# Autodesk Inventor assembly: LongAxisCradle
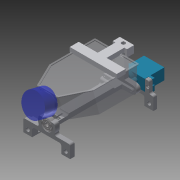
[picture p0: Inventor's stored thumbnail of the model, 180x180]
Saved by Autodesk Inventor 2014 SP1 (Build 180222100, 222)
## iProperties
Created: 2017-05-20
Part Number: LongAxisCradle
Document SubType Name: Assembly
Designer: danielsikar
Author: danielsikar
## Documents named in this file (9)
- C:\Users\danielsikar\Documents\Inventor\FlaskCradle\assemblies\LongAxisCradle.iam
- C:\Users\danielsikar\Documents\Inventor\FlaskCradle\parts\Flask.ipt
- C:\Users\danielsikar\Documents\Inventor\FlaskCradle\assemblies\ServoAndHorn.iam
- C:\Users\danielsikar\Documents\Inventor\FlaskCradle\parts\Bearing-605zz.ipt
- C:\Users\danielsikar\Documents\Inventor\FlaskCradle\parts\LongAxisShaft.ipt
- C:\Users\danielsikar\Documents\Inventor\FlaskCradle\parts\LongAxisTopClamp.ipt
- C:\Users\danielsikar\Documents\Inventor\FlaskCradle\parts\LongAxisServoSupport.ipt
- C:\Users\danielsikar\Documents\Inventor\FlaskCradle\parts\BearingSupport.ipt
- C:\Users\danielsikar\Documents\Inventor\FlaskCradle\parts\BaseSlat.ipt
## Components (8 placed, 8 different names)
1. Flask:1 — Mate:1, Mate:2, Mate:3, Mate:13, Mate:15, Mate:16, Mate:17
2. ServoAndHorn:1 [sub-assembly] — Mate:8, Mate:9, Mate:10, Mate:11, Mate:12, Mate:13, Mate:18, Mate:19, Mate:20
3. Bearing-605zz:1 — Mate:6, Mate:7, Flush:6
4. LongAxisShaft:1 — Mate:10, Mate:11, Mate:12
5. LongAxisTopClamp:1 — Mate:15, Mate:16, Mate:17
6. LongAxisServoSupport:1 — Mate:18, Mate:19, Mate:20, Mate:21, Mate:22, Mate:23
7. BearingSupport:1 — Flush:5, Flush:6
8. BaseSlat:1 — Mate:21, Mate:22, Mate:23
## Relationships (28: Mate 22, Flush 6)
- Mate:1: Flask:1
- Mate:2: Flask:1
- Mate:3: Flask:1
- Flush:1 (-3.5 mm)
- Flush:2 (24.85 mm)
- Mate:4
- Mate:5
- Flush:3 (-78 mm)
- Mate:6: Bearing-605zz:1
- Mate:7: Bearing-605zz:1
- Mate:8 (-6.25 mm): ServoAndHorn:1
- Mate:9: ServoAndHorn:1
- Mate:10: ServoAndHorn:1 ↔ LongAxisShaft:1
- Mate:11: ServoAndHorn:1 ↔ LongAxisShaft:1
- Mate:12: ServoAndHorn:1 ↔ LongAxisShaft:1
- Mate:13 (3 mm): Flask:1 ↔ ServoAndHorn:1
- Mate:15: Flask:1 ↔ LongAxisTopClamp:1
- Mate:16 (15 mm): Flask:1 ↔ LongAxisTopClamp:1
- Mate:17 (0.2 mm): Flask:1 ↔ LongAxisTopClamp:1
- Mate:18: ServoAndHorn:1 ↔ LongAxisServoSupport:1
- Mate:19: ServoAndHorn:1 ↔ LongAxisServoSupport:1
- Mate:20: ServoAndHorn:1 ↔ LongAxisServoSupport:1
- Flush:4 (-11 mm)
- Flush:5: BearingSupport:1
- Flush:6: Bearing-605zz:1 ↔ BearingSupport:1
- Mate:21: LongAxisServoSupport:1 ↔ BaseSlat:1
- Mate:22: LongAxisServoSupport:1 ↔ BaseSlat:1
- Mate:23: LongAxisServoSupport:1 ↔ BaseSlat:1
